# Autodesk Inventor assembly: ASY DUMMY TANK
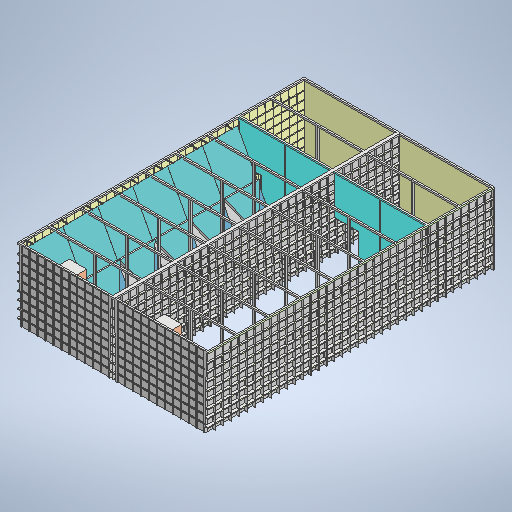
[picture p0: Inventor's stored thumbnail of the model, 512x512]
Saved by Autodesk Inventor 2026.2 (Build 302298000, 298)
## iProperties
Created: 2026-07-16
Part Number: ASY DUMMY TANK
Document SubType Name: Assembly
Designer: admin
Author: admin
## Documents named in this file (3)
- C:\Users\admin\Documents\Inventor\GBK-Gubkinskiy\dummy\ASY DUMMY TANK.iam
- C:\Users\admin\Documents\Inventor\GBK-Gubkinskiy\GBK overall model.ipt
- C:\Users\admin\Documents\Inventor\GBK-Gubkinskiy\dummy\Pocket.ipt
## Components (7 placed, 2 different names)
1. GBK overall model:1 — Mate:1, Mate:2, Flush:1
2. Pocket:1 — Mate:1, Mate:2, Flush:1
3. Pocket:2
4. Pocket:3
5. Pocket:4
6. Pocket:5
7. Pocket:6
## Component patterns: (6 elements, first: Pocket:1)
## Relationships (3: Mate 2, Flush 1)
- Mate:1: GBK overall model:1 ↔ Pocket:1
- Mate:2: GBK overall model:1 ↔ Pocket:1
- Flush:1: GBK overall model:1 ↔ Pocket:1
